# Autodesk Inventor assembly: ASY GBK 3130 central wall shield 3
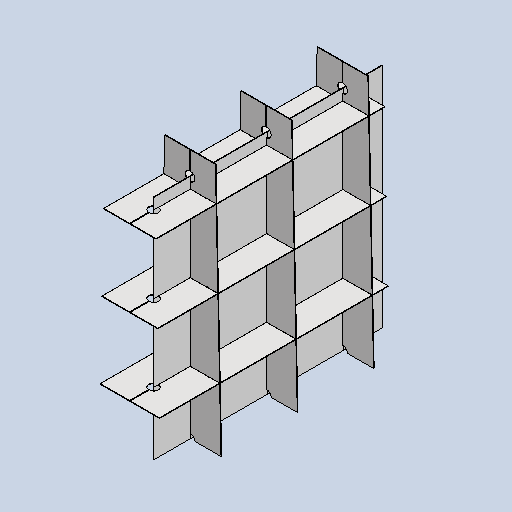
[picture p0: Inventor's stored thumbnail of the model, 512x512]
Saved by Autodesk Inventor 2026.2 (Build 302298010, 298A)
## iProperties
Created: 2026-05-19
Part Number: ASY GBK 3130 central wall shield 3
Document SubType Name: Assembly
Designer: pokla
Mass: 174041 g
Surface Area: 113034 cm^2
Volume: 22170.8 cm^3
Density: 7.85 g/cm^3
Author: admin
## Documents named in this file (8)
- C:\Users\admin\Documents\Inventor\GBK-Gubkinskiy\ASY GBK 3130 central wall shield 3.iam
- C:\Users\admin\Documents\Inventor\GBK-Gubkinskiy\GBK 0101 main rib.ipt
- C:\Users\admin\Documents\Inventor\GBK-Gubkinskiy\GBK 3133 shield 3.ipt
- C:\Users\admin\Documents\Inventor\GBK-Gubkinskiy\GBK 3112 central main rib_CPY1.ipt
- GBK 3112 central main rib_CPY1.ipt
- C:\Users\admin\Documents\Inventor\GBK-Gubkinskiy\GBK 3113 stringer 1.ipt
- C:\Users\admin\Documents\Inventor\GBK-Gubkinskiy\GBK 3114 stringer 2.ipt
- C:\Users\admin\Documents\Inventor\GBK-Gubkinskiy\GBK 3115 stringer 3.ipt
## Components (13 placed, 5 different names)
1. GBK 3113 stringer 1.ipt:1 — Rigid:1
2. GBK 3133 shield 3.ipt:1 — Mate:1, Flush:1, Mate:2, Flush:5, Flush:3, Mate:5, Flush:2, Mate:4
3. GBK 3114 stringer 2.ipt:1 — Rigid:2
4. GBK 3115 stringer 3.ipt:1 — Rigid:3
5. GBK 3113 stringer 1.ipt:2 — Rigid:6
6. GBK 3114 stringer 2.ipt:2 — Rigid:5
7. GBK 3115 stringer 3.ipt:2 — Rigid:6
8. GBK 3112 central main rib_CPY1.ipt:1 — Flush:5, Flush:3, Mate:5, Flush:4, Rigid:3, Rigid:2, Rigid:1
9. GBK 3112 central main rib_CPY1.ipt:2
10. GBK 3112 central main rib_CPY1.ipt:3
11. GBK 3112 central main rib_CPY1.ipt:4 — Flush:2, Mate:4, Flush:4, Rigid:6, Rigid:5, Rigid:6
12. GBK 3112 central main rib_CPY1.ipt:5
13. GBK 3112 central main rib_CPY1.ipt:6
## Component patterns: (3 elements, first: GBK 3112 central main rib_CPY1.ipt:1), (3 elements, first: GBK 3112 central main rib_CPY1.ipt:4)
## Relationships (15: WeldJoint 6, Flush 5, Mate 4)
- Mate:1: GBK 3133 shield 3.ipt:1
- Flush:1: GBK 3133 shield 3.ipt:1
- Mate:2: GBK 3133 shield 3.ipt:1
- Flush:5 (254 mm): GBK 3133 shield 3.ipt:1 ↔ GBK 3112 central main rib_CPY1.ipt:1
- Flush:3: GBK 3133 shield 3.ipt:1 ↔ GBK 3112 central main rib_CPY1.ipt:1
- Mate:5: GBK 3133 shield 3.ipt:1 ↔ GBK 3112 central main rib_CPY1.ipt:1
- Flush:2: GBK 3133 shield 3.ipt:1 ↔ GBK 3112 central main rib_CPY1.ipt:4
- Mate:4: GBK 3133 shield 3.ipt:1 ↔ GBK 3112 central main rib_CPY1.ipt:4
- Flush:4: GBK 3112 central main rib_CPY1.ipt:1 ↔ GBK 3112 central main rib_CPY1.ipt:4
- Rigid:3 [WeldJoint] (4 mm): GBK 3115 stringer 3.ipt:1 ↔ GBK 3112 central main rib_CPY1.ipt:1
- Rigid:2 [WeldJoint] (4 mm): GBK 3114 stringer 2.ipt:1 ↔ GBK 3112 central main rib_CPY1.ipt:1
- Rigid:1 [WeldJoint] (4 mm): GBK 3113 stringer 1.ipt:1 ↔ GBK 3112 central main rib_CPY1.ipt:1
- Rigid:6 [WeldJoint] (4 mm): GBK 3113 stringer 1.ipt:2 ↔ GBK 3112 central main rib_CPY1.ipt:4
- Rigid:5 [WeldJoint] (4 mm): GBK 3114 stringer 2.ipt:2 ↔ GBK 3112 central main rib_CPY1.ipt:4
- Rigid:6 [WeldJoint] (4 mm): GBK 3115 stringer 3.ipt:2 ↔ GBK 3112 central main rib_CPY1.ipt:4
## Named parameters: основание_длина_нижнего = 200 mm, основание_длина_верхнего = 100 mm, стрингер_глубина_1 = 190.70056 mm, стрингер_глубина_2 = 179.35977 mm, стрингер_глубина_3 = 168.01899 mm, стрингер_глубина_4 = 156.6782 mm, стрингер_глубина_5 = 145.33742 mm, стрингер_глубина_6 = 133.99663 mm, стрингер_глубина_7 = 122.65585 mm, стрингер_глубина_8 = 111.31507 mm, Лист_ширина = 1480 mm, ребро_усилителей = 60 mm, паз_под_стрингер_глубина = 70 mm, паз_под_стрингер_толщина = 5 mm, отступ_от_пола_до_первого_стрингера = 410 mm, шаг_стрингеров = 500 mm, радиус_выреза_под_сварку = 30 mm, нахлест_шпангоутов_1_2 = 150 mm, нахлест_шпангоутов_2_3 = 120 mm, Стрингер_длина = 1489.5 mm, Лист_длина = 2980 mm, Шаг_шпангоутов = 496.66667 mm
